# Autodesk Inventor assembly: assembly of 13 and 2
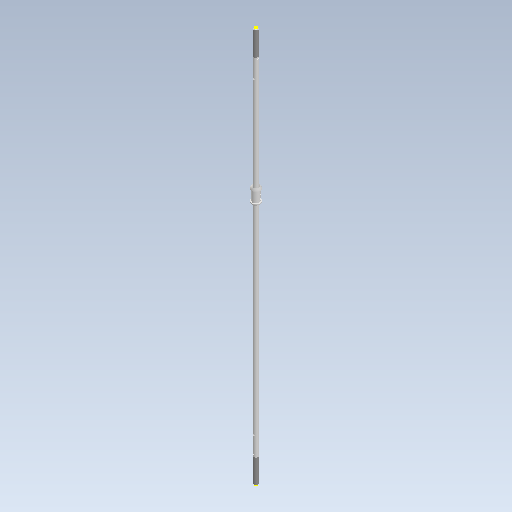
[picture p0: Inventor's stored thumbnail of the model, 512x512]
Saved by Autodesk Inventor 2020 (Build 240168000, 168)
## iProperties
Created: 2019-06-12
Part Number: assembly of 13 and 2
Document SubType Name: Weldment
Designer: ColinP
Weld Material: Welded Aluminum-6061
Author: ColinP
## Documents named in this file (4)
- C:\Users\ColinP\Documents\Inventor\igor\assembly of 13 and 2.iam
- C:\Users\ColinP\Documents\Inventor\igor\burner_rod_1or3.ipt
- C:\Users\ColinP\Documents\Inventor\igor\burder_rod_2.ipt
- C:\Users\ColinP\Documents\Inventor\igor\eyelet.ipt
## Components (5 placed, 3 different names)
1. burner_rod_1or3:1 — Insert:1
2. burner_rod_1or3:2 — Insert:2
3. burder_rod_2:1 — Insert:1, Insert:2, Mate:5
4. eyelet:5
5. eyelet:6 — Mate:5
## Relationships (4: Insert 2, RevoluteJoint 1, Mate 1)
- Insert:1: burner_rod_1or3:1 ↔ burder_rod_2:1
- Insert:2: burner_rod_1or3:2 ↔ burder_rod_2:1
- [RevoluteJoint]: eyelet:5 ↔ eyelet:6
- Mate:5: burder_rod_2:1 ↔ eyelet:6
## Named parameters: d12_d9 = 0 mm, d13_d10 = 92.356271 deg
